# Autodesk Inventor assembly: ECoG holder_2p1
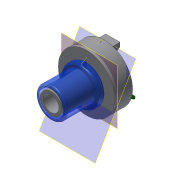
[picture p0: Inventor's stored thumbnail of the model, 180x180]
Saved by Autodesk Inventor 2014 (Build 180170000, 170)
## iProperties
Created: 2016-08-28
Part Number: ECoG holder_2p1
Document SubType Name: Assembly
Designer: Camilo
Author: Camilo
## Documents named in this file (8)
- Z:\Github\AgingTests\3D parts\ECoG holder_2p0\ECoG holder_2p1.iam
- Z:\Github\AgingTests\3D parts\ECoG holder\flaskPort.ipt
- Z:\Github\AgingTests\3D parts\ECoG holder_2p0\ECoG_holder_2p1.ipt
- Z:\Github\AgingTests\3D parts\ECoG holder_2p0\32ch_ECoG_assembled.iam
- Z:\Github\AgingTests\3D parts\ECoG holder_2p0\PTFEFilter_clamp.ipt
- Z:\Github\AgingTests\3D parts\ECoG holder_2p0\spaceFiller.ipt
- Z:\Github\AgingTests\3D parts\ECoG holder_2p0\spaceFiller_MIR1.ipt
- Z:\Github\AgingTests\3D parts\ECoG holder_2p0\PTFEFilter_clamp_MIR.ipt
## Components (7 placed, 7 different names)
1. flaskPort:1 — Mate:1, Flush:3, Mate:2, Flush:4
2. ECoG_holder_2p1:1 — Flush:4, Mate:3, Mate:4, Flush:5, Flush:6, Flush:7, Flush:8, Flush:9
3. 32ch_ECoG_assembled:1 [sub-assembly] — Mate:3, Mate:4, Flush:5
4. PTFEFilter_clamp:1 — Flush:6, Flush:7
5. spaceFiller:1 — Flush:8, Flush:9
6. spaceFiller_MIR1:1
7. PTFEFilter_clamp_MIR:1
## Relationships (11: Flush 7, Mate 4)
- Mate:1: flaskPort:1
- Flush:3: flaskPort:1
- Mate:2: flaskPort:1
- Flush:4: flaskPort:1 ↔ ECoG_holder_2p1:1
- Mate:3: ECoG_holder_2p1:1 ↔ 32ch_ECoG_assembled:1
- Mate:4: ECoG_holder_2p1:1 ↔ 32ch_ECoG_assembled:1
- Flush:5: ECoG_holder_2p1:1 ↔ 32ch_ECoG_assembled:1
- Flush:6: ECoG_holder_2p1:1 ↔ PTFEFilter_clamp:1
- Flush:7: ECoG_holder_2p1:1 ↔ PTFEFilter_clamp:1
- Flush:8: ECoG_holder_2p1:1 ↔ spaceFiller:1
- Flush:9: ECoG_holder_2p1:1 ↔ spaceFiller:1
